# Autodesk Inventor assembly: Тестовая серва
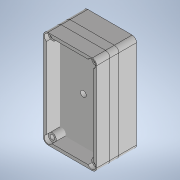
[picture p0: Inventor's stored thumbnail of the model, 180x180]
Saved by Autodesk Inventor 2020 (Build 240168000, 168)
## iProperties
Created: 2021-09-05
Part Number: Тестовая серва
Document SubType Name: Assembly
Designer: Антон
Author: Антон
## Documents named in this file (3)
- D:\Project\Robots\FutureEngineersViolet\3D-models\RRO 2021 Mk. IV\Тестовая серва\Тестовая серва.iam
- D:\Project\Robots\FutureEngineersViolet\3D-models\RRO 2021 Mk. IV\Тестовая серва\Основание сервы.ipt
- D:\Project\Robots\FutureEngineersViolet\3D-models\RRO 2021 Mk. IV\Тестовая серва\Голова сервы.ipt
## Components (2 placed, 2 different names)
1. Основание сервы:1 — Жесткий:1
2. Голова сервы:1 — Жесткий:1
## Relationships (1: WeldJoint 1)
- Жесткий:1 [WeldJoint]: Основание сервы:1 ↔ Голова сервы:1
